# Autodesk Inventor assembly: RollingSquareC1
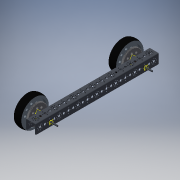
[picture p0: Inventor's stored thumbnail of the model, 180x180]
Saved by Autodesk Inventor 2016 (Build 200138000, 138)
## iProperties
Created: 2015-08-30
Part Number: RollingSquareC1
Document SubType Name: Assembly
Designer: Tim
Author: Tim
## Documents named in this file (6)
- C:\Users\Tim\Documents\GitHub\phi_robotics\3d-models\FTC_Tetrix_KOP_Block_Party\Tim Bloot Designs\RollingSquareC1.iam
- C:\Users\Tim\Documents\GitHub\phi_robotics\3d-models\FTC_Tetrix_KOP_Block_Party\Tetrix_Kit_FTC\Autodesk Inventor Files\tetrix_c_channel-5.ipt
- C:\Users\Tim\Documents\GitHub\phi_robotics\3d-models\FTC_Tetrix_KOP_Block_Party\Tetrix_Kit_FTC\Autodesk Inventor Files\tetrix_bushing.ipt
- C:\Users\Tim\Documents\GitHub\phi_robotics\3d-models\FTC_Tetrix_KOP_Block_Party\Tetrix_Kit_FTC\Autodesk Inventor Files\tetrix_axle.ipt
- C:\Users\Tim\Documents\GitHub\phi_robotics\3d-models\FTC_Tetrix_KOP_Block_Party\Tetrix_Kit_FTC\Autodesk Inventor Files\tetrix_739092_2012.iam
- C:\Users\Tim\Documents\GitHub\phi_robotics\3d-models\FTC_Tetrix_KOP_Block_Party\WheelNGear.iam
## Components (11 placed, 5 different names)
1. tetrix_c_channel-5:1 — Rotational:3, Rotational:4, Rotational:6, Rotational:7
2. tetrix_bushing:3 — Rotational:3
3. tetrix_bushing:4 — Rotational:4, Rotational:5
4. tetrix_axle:1 — Rotational:5, Rigid:1, Rigid:7
5. tetrix_739092_2012:1 [sub-assembly] — Rigid:1
6. tetrix_bushing:5 — Rotational:6
7. tetrix_bushing:6 — Rotational:7, Rotational:8
8. tetrix_axle:2 — Rigid:2, Rotational:8, Rigid:6
9. tetrix_739092_2012:2 [sub-assembly] — Rigid:2
10. WheelNGear:3 [sub-assembly] — Rigid:7
11. WheelNGear:4 [sub-assembly] — Rigid:6
## Relationships (10: RevoluteJoint 6, WeldJoint 4)
- Rotational:3 [RevoluteJoint]: tetrix_c_channel-5:1 ↔ tetrix_bushing:3
- Rotational:4 [RevoluteJoint]: tetrix_c_channel-5:1 ↔ tetrix_bushing:4
- Rotational:5 [RevoluteJoint] (-25 mm): tetrix_bushing:4 ↔ tetrix_axle:1
- Rigid:1 [WeldJoint] (-19.2 mm): tetrix_axle:1 ↔ tetrix_739092_2012:1
- Rotational:6 [RevoluteJoint]: tetrix_c_channel-5:1 ↔ tetrix_bushing:5
- Rotational:7 [RevoluteJoint]: tetrix_c_channel-5:1 ↔ tetrix_bushing:6
- Rigid:2 [WeldJoint] (-19.2 mm): tetrix_axle:2 ↔ tetrix_739092_2012:2
- Rotational:8 [RevoluteJoint] (25 mm): tetrix_bushing:6 ↔ tetrix_axle:2
- Rigid:6 [WeldJoint] (-1 mm): tetrix_axle:2 ↔ WheelNGear:4
- Rigid:7 [WeldJoint] (-1 mm): tetrix_axle:1 ↔ WheelNGear:3
## Named parameters: d21_d16 = -19.2 mm
